# Autodesk Inventor assembly: Suspenion_Arm_Assembly_V2
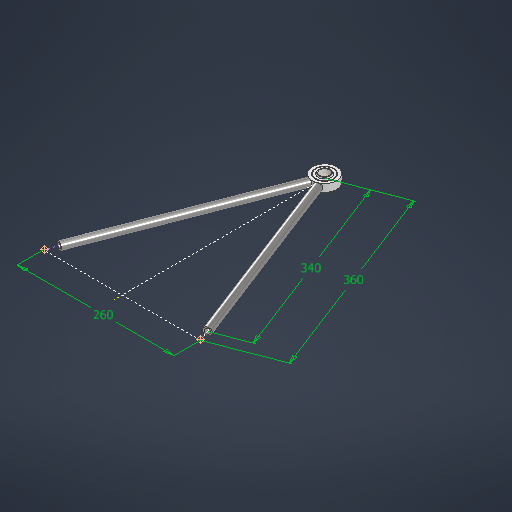
[picture p0: Inventor's stored thumbnail of the model, 512x512]
Saved by Autodesk Inventor 2026.1 (Build 301233000, 233)
## iProperties
Created: 2026-09-19
Part Number: Suspenion_Arm_Assembly_V2
Document SubType Name: Assembly
Designer: share
Author: share
## iProperties of the stored document MemberDocs/xIbebkxihE0miwt5rDgfrir3fBc
Created: 2026-09-19
Part Number: Suspenion_Arm_Assembly_V2
Document SubType Name: Assembly
Designer: share
Author: share
## iProperties of the stored document MemberDocs/x3ppwbxjtNsr3h3a3YmdzjtaqHa
Created: 2026-09-19
Part Number: Suspenion_Arm_Assembly_V2
Document SubType Name: Assembly
Designer: share
Author: share
## iProperties of the stored document MemberDocs/xP0ibiad1Fczjh2g1I2f14qfxOa
Created: 2026-09-19
Part Number: Suspenion_Arm_Assembly_V2
Document SubType Name: Assembly
Designer: share
Author: share
## iProperties of the stored document MemberDocs/xW3cjvtjaBcbywddnEbiznnn2Ca
Created: 2026-09-19
Part Number: Suspenion_Arm_Assembly_V2
Document SubType Name: Assembly
Designer: share
Author: share
## Documents named in this file (12)
- C:\Users\W Ahmad\Desktop\FSAE- Summer 2026 Project\FSAE CAD\GOGO_KART_FSAE\Suspension\Suspension_Arm_V2\Suspenion_Arm_Assembly_V2.iam
- C:\Users\share\OneDrive\Documents\Personal Projects\GOGO Kart\CAD\GOGO_KART_FSAE\Suspension\Suspension_Arm_V2\Suspenion_Arm_Outline_Sketch_V2.ipt
- C:\Users\share\OneDrive\Documents\Personal Projects\GOGO Kart\CAD\GOGO_KART_FSAE\Suspension\Suspension_Arm_V2\Outboard_Bearing_Housing.ipt
- C:\Users\share\OneDrive\Documents\Personal Projects\GOGO Kart\CAD\GOGO_KART_FSAE\Suspension\Suspension_Arm_V2\Suspenion_Arm_Assembly_V2\Frame\Frame 1789855613208.iam
- C:\Users\share\OneDrive\Documents\Personal Projects\GOGO Kart\CAD\GOGO_KART_FSAE\Suspension\Suspension_Arm_V2\63195K75_Swivel Joint (1).ipt
- C:\Users\share\OneDrive\Documents\Personal Projects\GOGO Kart\CAD\GOGO_KART_FSAE\Suspension\Suspension_Arm_V2\60645K141_Ball Joint Rod End\60645K141_Ball Joint Rod End\60645K141_Ball Joint Rod End.ipt
- C:\Users\share\OneDrive\Documents\Inventor\Content Center Files\R2026\en-US\ISO 4035(2)\ISO 4035 - M10 - ISO.ipt
- C:\Users\W Ahmad\Desktop\FSAE- Summer 2026 Project\FSAE CAD\GOGO_KART_FSAE\Suspension\Suspension_Arm_V2\Suspenion_Arm_Outline_Sketch_V2.ipt
- C:\Users\W Ahmad\Desktop\FSAE- Summer 2026 Project\FSAE CAD\GOGO_KART_FSAE\Suspension\Suspension_Arm_V2\Outboard_Bearing_Housing.ipt
- C:\Users\W Ahmad\Desktop\FSAE- Summer 2026 Project\FSAE CAD\GOGO_KART_FSAE\Suspension\Suspension_Arm_V2\63195K75_Swivel Joint (1).ipt
- C:\Users\W Ahmad\Desktop\FSAE- Summer 2026 Project\FSAE CAD\GOGO_KART_FSAE\Suspension\Suspension_Arm_V2\60645K141_Ball Joint Rod End\60645K141_Ball Joint Rod End\60645K141_Ball Joint Rod End.ipt
- C:\Users\W Ahmad\Desktop\FSAE- Summer 2026 Project\FSAE CAD\GOGO_KART_FSAE\Suspension\Suspension_Arm_V2\Suspenion_Arm_Assembly_V2_Member.ipt
## Components (8 placed, 6 different names)
1. Suspenion_Arm_Outline_Sketch_V2:1 — Flush:1, Flush:2, Flush:3, Mate:3, Mate:7, Mate:8, Mate:9, Mate:10
2. Outboard_Bearing_Housing:1 — Mate:2, Mate:3, Mate:6
3. Frame 1789855613208:1 [sub-assembly] — Insert:1, Insert:2
4. 63195K75_Swivel Joint (1):1 — Mate:5, Mate:6
5. 60645K141_Ball Joint Rod End:1 — Mate:7, Mate:8, Mate:11
6. 60645K141_Ball Joint Rod End:2 — Mate:9, Mate:10, Mate:12
7. ISO 4035 M10:1 — Insert:1
8. ISO 4035 M10:2 — Insert:2
## Relationships (15: Mate 10, Flush 3, Insert 2)
- Flush:1: Suspenion_Arm_Outline_Sketch_V2:1
- Flush:2: Suspenion_Arm_Outline_Sketch_V2:1
- Flush:3: Suspenion_Arm_Outline_Sketch_V2:1
- Mate:2: Outboard_Bearing_Housing:1
- Mate:3: Suspenion_Arm_Outline_Sketch_V2:1 ↔ Outboard_Bearing_Housing:1
- Mate:5: 63195K75_Swivel Joint (1):1
- Mate:6: Outboard_Bearing_Housing:1 ↔ 63195K75_Swivel Joint (1):1
- Mate:7: Suspenion_Arm_Outline_Sketch_V2:1 ↔ 60645K141_Ball Joint Rod End:1
- Mate:8: Suspenion_Arm_Outline_Sketch_V2:1 ↔ 60645K141_Ball Joint Rod End:1
- Mate:9: Suspenion_Arm_Outline_Sketch_V2:1 ↔ 60645K141_Ball Joint Rod End:2
- Mate:10: Suspenion_Arm_Outline_Sketch_V2:1 ↔ 60645K141_Ball Joint Rod End:2
- Mate:11: 60645K141_Ball Joint Rod End:1
- Mate:12: 60645K141_Ball Joint Rod End:2
- Insert:1: Frame 1789855613208:1 ↔ ISO 4035 M10:1
- Insert:2: Frame 1789855613208:1 ↔ ISO 4035 M10:2
